# Autodesk Inventor assembly: Assembly2
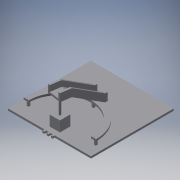
[picture p0: Inventor's stored thumbnail of the model, 180x180]
Saved by Autodesk Inventor 2018 (Build 220112000, 112)
## iProperties
Created: 2018-04-30
Part Number: Assembly2
Document SubType Name: Assembly
Designer: Administrator
Author: Administrator
## Documents named in this file (11)
- E:\Folders\School\10th Grade\Digital Electronics\Final Project\CAD Designs\Assembly2.iam
- E:\Folders\School\10th Grade\Digital Electronics\Final Project\CAD Designs\Part7.ipt
- E:\Folders\School\10th Grade\Digital Electronics\Final Project\CAD Designs\Part8.ipt
- E:\Folders\School\10th Grade\Digital Electronics\Final Project\CAD Designs\Part9.ipt
- E:\Folders\School\10th Grade\Digital Electronics\Final Project\CAD Designs\Part10.ipt
- E:\Folders\School\10th Grade\Digital Electronics\Final Project\CAD Designs\Part11.ipt
- E:\Folders\School\10th Grade\Digital Electronics\Final Project\CAD Designs\Part12.ipt
- C:\Users\jerrywang\Documents\Part13.ipt
- C:\Users\jerrywang\Documents\Part14.ipt
- C:\Users\jerrywang\Documents\Part15.ipt
- C:\Users\jerrywang\Documents\Part16.ipt
## Components (15 placed, 10 different names)
1. Part7:1 — Flush:10, Mate:1, Flush:17, Mate:3, Flush:21, Mate:9, Insert:1
2. Part8:2 — Flush:1, Flush:4, Flush:7, Mate:1, Flush:18, Flush:19, Mate:3
3. Part8:3 — Flush:1, Flush:3, Flush:4, Flush:7, Flush:12, Flush:13, Flush:15
4. Part8:4 — Flush:3, Flush:10, Flush:11, Flush:14, Flush:18, Flush:19, Flush:20
5. Part9:1 — Flush:11, Flush:12, Flush:13, Flush:16, Mate:2
6. Part10:1 — Flush:14, Flush:15, Flush:16
7. Part11:1 — Flush:17, Mate:2, Flush:20, Mate:4, Mate:5, Mate:6, Mate:7, Flush:22, Mate:8, Flush:23
8. Part12:1 — Mate:4, Mate:5, Flush:21
9. Part12:2 — Mate:6, Mate:7, Flush:22
10. Part12:3 — Mate:8, Mate:9, Flush:23
11. Part13:1 — Flush:27, Flush:28, Flush:29, Flush:30, Mate:10, Flush:31
12. Part14:1 — Insert:1, Insert:2
13. Part15:1 — Flush:24, Flush:25, Flush:26, Flush:27, Flush:28, Flush:31, Insert:2
14. Part13:2 — Flush:24, Flush:25, Flush:26
15. Part16:1 — Flush:29, Flush:30, Mate:10
## Relationships (38: Flush 26, Mate 10, Insert 2)
- Flush:1: Part8:2 ↔ Part8:3
- Flush:3: Part8:3 ↔ Part8:4
- Flush:4: Part8:2 ↔ Part8:3
- Flush:7: Part8:2 ↔ Part8:3
- Flush:10: Part7:1 ↔ Part8:4
- Mate:1: Part7:1 ↔ Part8:2
- Flush:11: Part8:4 ↔ Part9:1
- Flush:12: Part8:3 ↔ Part9:1
- Flush:13: Part8:3 ↔ Part9:1
- Flush:14: Part8:4 ↔ Part10:1
- Flush:15: Part8:3 ↔ Part10:1
- Flush:16: Part9:1 ↔ Part10:1
- Flush:17 (12.7 mm): Part7:1 ↔ Part11:1
- Mate:2 (63.5 mm): Part9:1 ↔ Part11:1
- Flush:18: Part8:2 ↔ Part8:4
- Flush:19: Part8:2 ↔ Part8:4
- Mate:3: Part7:1 ↔ Part8:2
- Flush:20 (12.7 mm): Part8:4 ↔ Part11:1
- Mate:4: Part11:1 ↔ Part12:1
- Mate:5: Part11:1 ↔ Part12:1
- Flush:21: Part7:1 ↔ Part12:1
- Mate:6: Part11:1 ↔ Part12:2
- Mate:7: Part11:1 ↔ Part12:2
- Flush:22: Part11:1 ↔ Part12:2
- Mate:8: Part11:1 ↔ Part12:3
- Mate:9: Part7:1 ↔ Part12:3
- Flush:23: Part11:1 ↔ Part12:3
- Insert:1: Part7:1 ↔ Part14:1
- Flush:24: Part15:1 ↔ Part13:2
- Flush:25: Part15:1 ↔ Part13:2
- Flush:26: Part15:1 ↔ Part13:2
- Flush:27: Part13:1 ↔ Part15:1
- Flush:28: Part13:1 ↔ Part15:1
- Flush:29: Part13:1 ↔ Part16:1
- Flush:30: Part13:1 ↔ Part16:1
- Mate:10: Part13:1 ↔ Part16:1
- Flush:31: Part13:1 ↔ Part15:1
- Insert:2: Part14:1 ↔ Part15:1
